# Autodesk Inventor assembly: złożenie gąsienicy lewej
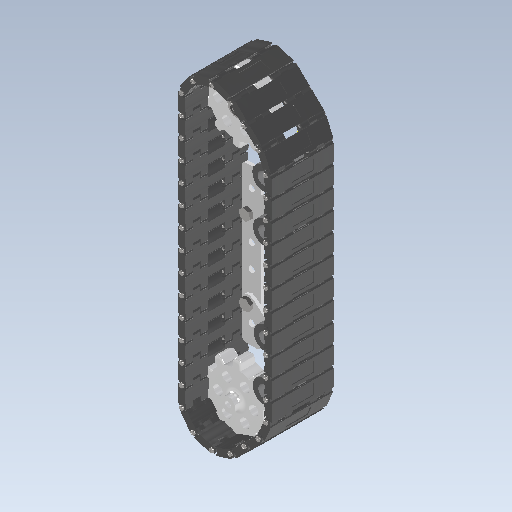
[picture p0: Inventor's stored thumbnail of the model, 512x512]
Saved by Autodesk Inventor 2021 (Build 250183000, 183)
## iProperties
Created: 2021-06-19
Part Number: złożenie gąsienicy lewej
Document SubType Name: Assembly
Designer: Łukasz
Author: Łukasz
## Documents named in this file (14)
- E:\GITHUB_Czołg\Szybki-Czolg-antyRadziecki\złożenie gąsienicy lewej.iam
- E:\GITHUB_Czołg\Szybki-Czolg-antyRadziecki\gąsienica.ipt
- E:\GITHUB_Czołg\Szybki-Czolg-antyRadziecki\koło napędowe.ipt
- E:\GITHUB_Czołg\Szybki-Czolg-antyRadziecki\koło łożyskowane.ipt
- E:\GITHUB_Czołg\Szybki-Czolg-antyRadziecki\dystans łożyska.ipt
- E:\GITHUB_Czołg\Szybki-Czolg-antyRadziecki\mocowanie zawieszenia.ipt
- C:\Users\Łukasz\Documents\Inventor\Content Center Files\R2021\en-US\BS EN ISO 7045 H\EN ISO 7045 - M3 x 30 - 4.8 - H(1).ipt
- E:\GITHUB_Czołg\Szybki-Czolg-antyRadziecki\zawieszenie ramie.ipt
- C:\Users\Łukasz\Documents\Inventor\Content Center Files\R2021\en-US\BS 292 (I)\BS 292 Part 1 - 608 - 8 x 22 x 7.ipt
- E:\GITHUB_Czołg\Szybki-Czolg-antyRadziecki\zawieszenie ramie 2.ipt
- C:\Users\Łukasz\Documents\Inventor\Content Center Files\R2021\en-US\BS EN ISO 4017\BS EN ISO 4017 - M8 x 20BS EN.ipt
- C:\Users\Łukasz\Documents\Inventor\Content Center Files\R2021\en-US\AS 1112 (2)\AS 1112 - M8  Type 8.ipt
- C:\Users\Łukasz\Documents\Inventor\Content Center Files\R2021\en-US\AS 1427(02)\AS 1427 - M8 x 25(2).ipt
- E:\GITHUB_Czołg\Szybki-Czolg-antyRadziecki\kółko zawieszenia.ipt
## Components (153 placed, 13 different names)
1. gąsienica:1 — Rotational:1, Angle:1, Rotational:6, Angle:6, Rotational:66, Rotational:77
2. gąsienica:2 — Rotational:1, Angle:1, Rotational:2, Angle:2, Flush:4, Rotational:65, Rotational:78
3. gąsienica:3 — Rotational:5, Angle:5, Rotational:7, Angle:8, Rotational:61, Rotational:82
4. gąsienica:4 — Rotational:3, Angle:3, Rotational:4, Angle:4, Rotational:63, Rotational:80
5. gąsienica:5 — Rotational:2, Angle:2, Rotational:3, Angle:3, Mate:1, Flush:1, Rotational:64, Rotational:79
6. gąsienica:6 — Rotational:6, Angle:6, Rotational:9, Angle:7, Rotational:67, Rotational:76
7. gąsienica:7 — Rotational:4, Angle:4, Rotational:5, Angle:5, Rotational:62, Rotational:81
8. gąsienica:8 — Rotational:7, Rotational:8, Angle:8, Angle:9, Rotational:60, Rotational:83
9. gąsienica:9 — Rotational:8, Angle:9, Rotational:31, Angle:28, Rotational:59, Rotational:84
10. gąsienica:10 — Rotational:9, Angle:7, Rotational:10, Angle:10, Rotational:68, Rotational:113
11. koło napędowe:1 — Mate:1, Flush:1, Flush:3, Mate:2, Mate:3, Flush:4, Flush:5, Flush:6, Mate:4
12. koło łożyskowane:1 — Flush:3, Mate:2, Mate:3, Insert:1, Insert:2, Insert:3
13. dystans łożyska:1 — Insert:1
14. BS 292: Part 1 (I) (Metric) 608 - 8 x 22 x 7:13 — Insert:2
15. BS 292: Part 1 (I) (Metric) 608 - 8 x 22 x 7:14 — Insert:3
16. gąsienica:11 — Rotational:10, Rotational:11, Angle:10, Angle:11, Rotational:69, Rotational:112
17. gąsienica:12 — Rotational:11, Angle:11, Rotational:12, Angle:12, Rotational:71, Rotational:111
18. gąsienica:13 — Rotational:13, Rotational:14, Angle:13, Angle:14, Rotational:72, Rotational:109
19. gąsienica:14 — Rotational:14, Angle:14, Rotational:15, Angle:15, Rotational:73, Rotational:108
20. gąsienica:15 — Rotational:15, Rotational:16, Angle:15, Angle:16, Rotational:74, Rotational:107
21. gąsienica:16 — Rotational:12, Rotational:13, Angle:12, Angle:13, Rotational:70, Rotational:110
22. gąsienica:17 — Rotational:16, Angle:16, Rotational:17, Angle:17, Rotational:75, Rotational:106
23. gąsienica:18 — Rotational:17, Rotational:18, Angle:17, Angle:18, Rotational:41, Rotational:105
24. gąsienica:19 — Rotational:18, Angle:18, Rotational:19, Angle:19, Rotational:40, Rotational:104
25. gąsienica:20 — Rotational:19, Rotational:20, Angle:19, Angle:20, Rotational:39, Rotational:103
26. gąsienica:21 — Rotational:20, Angle:20, Rotational:21, Angle:21, Rotational:42, Rotational:102
27. gąsienica:22 — Rotational:21, Rotational:22, Angle:21, Angle:22, Rotational:43, Rotational:101
28. gąsienica:23 — Rotational:22, Angle:22, Rotational:23, Angle:23, Rotational:44, Rotational:100
29. gąsienica:24 — Rotational:23, Rotational:24, Angle:23, Angle:24, Rotational:45, Rotational:99
30. gąsienica:25 — Rotational:24, Angle:24, Rotational:25, Angle:25, Rotational:46, Rotational:114
31. gąsienica:26 — Rotational:25, Rotational:26, Angle:25, Angle:26, Rotational:47, Rotational:96
32. gąsienica:27 — Rotational:26, Rotational:27, Angle:26, Angle:27, Rotational:48, Rotational:95
33. gąsienica:28 — Rotational:27, Angle:27, Rotational:37, Angle:36, Rotational:49, Rotational:94
34. gąsienica:29 — Rotational:29, Angle:30, Rotational:32, Angle:32, Rotational:56
35. gąsienica:30 — Rotational:29, Rotational:30, Angle:29, Angle:30, Rotational:57, Rotational:86
36. gąsienica:31 — Rotational:30, Rotational:31, Angle:28, Angle:29, Rotational:58, Rotational:85
37. gąsienica:32 — Rotational:32, Rotational:33, Angle:31, Angle:32, Rotational:55, Rotational:87
38. gąsienica:33 — Rotational:33, Angle:31, Rotational:34, Angle:33, Rotational:54, Rotational:88, Rotational:89
39. gąsienica:34 — Rotational:34, Rotational:36, Angle:33, Angle:34, Rotational:53, Rotational:90
40. gąsienica:35 — Rotational:35, Angle:35, Rotational:38, Angle:37, Rotational:51
41. gąsienica:36 — Rotational:35, Rotational:36, Angle:34, Angle:35, Rotational:52, Rotational:91
42. gąsienica:37 — Rotational:37, Angle:36, Rotational:38, Angle:37, Rotational:50, Rotational:92, Rotational:93
43. mocowanie zawieszenia:1 — Flush:5, Flush:6, Mate:4, Rotational:116, Rotational:125, Rotational:142, Rotational:144
44. BS EN ISO 7045 H - Metric M3 x 30 - 4.8 - H:1 — Rotational:39
45. BS EN ISO 7045 H - Metric M3 x 30 - 4.8 - H:2 — Rotational:40
46. BS EN ISO 7045 H - Metric M3 x 30 - 4.8 - H:3 — Rotational:83
47. BS EN ISO 7045 H - Metric M3 x 30 - 4.8 - H:4 — Rotational:82
48. BS EN ISO 7045 H - Metric M3 x 30 - 4.8 - H:5 — Rotational:75
49. BS EN ISO 7045 H - Metric M3 x 30 - 4.8 - H:6 — Rotational:74
50. BS EN ISO 7045 H - Metric M3 x 30 - 4.8 - H:7 — Rotational:73
51. BS EN ISO 7045 H - Metric M3 x 30 - 4.8 - H:8 — Rotational:72
52. BS EN ISO 7045 H - Metric M3 x 30 - 4.8 - H:9 — Rotational:71
53. BS EN ISO 7045 H - Metric M3 x 30 - 4.8 - H:10 — Rotational:70
54. BS EN ISO 7045 H - Metric M3 x 30 - 4.8 - H:11 — Rotational:69
55. BS EN ISO 7045 H - Metric M3 x 30 - 4.8 - H:12 — Rotational:68
56. BS EN ISO 7045 H - Metric M3 x 30 - 4.8 - H:13 — Rotational:67
57. BS EN ISO 7045 H - Metric M3 x 30 - 4.8 - H:14 — Rotational:66
58. BS EN ISO 7045 H - Metric M3 x 30 - 4.8 - H:15 — Rotational:65
59. BS EN ISO 7045 H - Metric M3 x 30 - 4.8 - H:16 — Rotational:64
60. BS EN ISO 7045 H - Metric M3 x 30 - 4.8 - H:17 — Rotational:63
61. BS EN ISO 7045 H - Metric M3 x 30 - 4.8 - H:18 — Rotational:62
62. BS EN ISO 7045 H - Metric M3 x 30 - 4.8 - H:19 — Rotational:61
63. BS EN ISO 7045 H - Metric M3 x 30 - 4.8 - H:20 — Rotational:60
64. BS EN ISO 7045 H - Metric M3 x 30 - 4.8 - H:21 — Rotational:59
65. BS EN ISO 7045 H - Metric M3 x 30 - 4.8 - H:22 — Rotational:58
66. BS EN ISO 7045 H - Metric M3 x 30 - 4.8 - H:23 — Rotational:57
67. BS EN ISO 7045 H - Metric M3 x 30 - 4.8 - H:24 — Rotational:56
68. BS EN ISO 7045 H - Metric M3 x 30 - 4.8 - H:25 — Rotational:54
69. BS EN ISO 7045 H - Metric M3 x 30 - 4.8 - H:26 — Rotational:52
70. BS EN ISO 7045 H - Metric M3 x 30 - 4.8 - H:27 — Rotational:53
71. BS EN ISO 7045 H - Metric M3 x 30 - 4.8 - H:28 — Rotational:55
72. BS EN ISO 7045 H - Metric M3 x 30 - 4.8 - H:29 — Rotational:51
73. BS EN ISO 7045 H - Metric M3 x 30 - 4.8 - H:30 — Rotational:50
74. BS EN ISO 7045 H - Metric M3 x 30 - 4.8 - H:31 — Rotational:49
75. BS EN ISO 7045 H - Metric M3 x 30 - 4.8 - H:32 — Rotational:48
76. BS EN ISO 7045 H - Metric M3 x 30 - 4.8 - H:33 — Rotational:47
77. BS EN ISO 7045 H - Metric M3 x 30 - 4.8 - H:34 — Rotational:46
78. BS EN ISO 7045 H - Metric M3 x 30 - 4.8 - H:35 — Rotational:45
79. BS EN ISO 7045 H - Metric M3 x 30 - 4.8 - H:36 — Rotational:44
80. BS EN ISO 7045 H - Metric M3 x 30 - 4.8 - H:37 — Rotational:43
81. BS EN ISO 7045 H - Metric M3 x 30 - 4.8 - H:38 — Rotational:42
82. BS EN ISO 7045 H - Metric M3 x 30 - 4.8 - H:39 — Rotational:41
83. BS EN ISO 7045 H - Metric M3 x 30 - 4.8 - H:40 — Rotational:76
84. BS EN ISO 7045 H - Metric M3 x 30 - 4.8 - H:41 — Rotational:77
85. BS EN ISO 7045 H - Metric M3 x 30 - 4.8 - H:42 — Rotational:78
86. BS EN ISO 7045 H - Metric M3 x 30 - 4.8 - H:43 — Rotational:79
87. BS EN ISO 7045 H - Metric M3 x 30 - 4.8 - H:44 — Rotational:80
88. BS EN ISO 7045 H - Metric M3 x 30 - 4.8 - H:45 — Rotational:81
89. BS EN ISO 7045 H - Metric M3 x 30 - 4.8 - H:46 — Rotational:84
90. BS EN ISO 7045 H - Metric M3 x 30 - 4.8 - H:47 — Rotational:85
91. BS EN ISO 7045 H - Metric M3 x 30 - 4.8 - H:48 — Rotational:86
92. BS EN ISO 7045 H - Metric M3 x 30 - 4.8 - H:49 — Rotational:87
93. BS EN ISO 7045 H - Metric M3 x 30 - 4.8 - H:50 — Rotational:88
94. BS EN ISO 7045 H - Metric M3 x 30 - 4.8 - H:51 — Rotational:89
95. BS EN ISO 7045 H - Metric M3 x 30 - 4.8 - H:52 — Rotational:90
96. BS EN ISO 7045 H - Metric M3 x 30 - 4.8 - H:53 — Rotational:91
97. BS EN ISO 7045 H - Metric M3 x 30 - 4.8 - H:54 — Rotational:92
98. BS EN ISO 7045 H - Metric M3 x 30 - 4.8 - H:55 — Rotational:93
99. BS EN ISO 7045 H - Metric M3 x 30 - 4.8 - H:56 — Rotational:94
100. BS EN ISO 7045 H - Metric M3 x 30 - 4.8 - H:57 — Rotational:95
101. BS EN ISO 7045 H - Metric M3 x 30 - 4.8 - H:58 — Rotational:96
102. BS EN ISO 7045 H - Metric M3 x 30 - 4.8 - H:60 — Rotational:114
103. BS EN ISO 7045 H - Metric M3 x 30 - 4.8 - H:61 — Rotational:99
104. BS EN ISO 7045 H - Metric M3 x 30 - 4.8 - H:62 — Rotational:100
105. BS EN ISO 7045 H - Metric M3 x 30 - 4.8 - H:63 — Rotational:101
106. BS EN ISO 7045 H - Metric M3 x 30 - 4.8 - H:64 — Rotational:102
107. BS EN ISO 7045 H - Metric M3 x 30 - 4.8 - H:65 — Rotational:103
108. BS EN ISO 7045 H - Metric M3 x 30 - 4.8 - H:66 — Rotational:104
109. BS EN ISO 7045 H - Metric M3 x 30 - 4.8 - H:67 — Rotational:105
110. BS EN ISO 7045 H - Metric M3 x 30 - 4.8 - H:68 — Rotational:106
111. BS EN ISO 7045 H - Metric M3 x 30 - 4.8 - H:69 — Rotational:107
112. BS EN ISO 7045 H - Metric M3 x 30 - 4.8 - H:70 — Rotational:108
113. BS EN ISO 7045 H - Metric M3 x 30 - 4.8 - H:71 — Rotational:109
114. BS EN ISO 7045 H - Metric M3 x 30 - 4.8 - H:72 — Rotational:110
115. BS EN ISO 7045 H - Metric M3 x 30 - 4.8 - H:73 — Rotational:113
116. BS EN ISO 7045 H - Metric M3 x 30 - 4.8 - H:74 — Rotational:111
117. BS EN ISO 7045 H - Metric M3 x 30 - 4.8 - H:75 — Rotational:112
118. zawieszenie ramie:1 — Rotational:116, Rotational:117, Rotational:119, Rotational:121
119. zawieszenie ramie:2 — Rotational:118, Rotational:122, Rotational:142, Rotational:143
120. AS 1427 - Metric M8 x 25:1 — Rigid:2
121. BS 292: Part 1 (I) (Metric) 608 - 8 x 22 x 7:5 — Rotational:126, Rigid:6, Rotational:137
122. zawieszenie ramie 2:1 — Rotational:117, Rotational:123, Rotational:126, Rotational:127, Rotational:128, Rotational:129
123. zawieszenie ramie 2:2 — Rotational:118, Rotational:130, Rotational:131, Rotational:132, Rotational:133, Rigid:10
124. BS EN ISO 4017 - Metric M8 x 20:1 — Rotational:119
125. BS EN ISO 4017 - Metric M8 x 20:2 — Rotational:122
126. BS EN ISO 4017 - Metric M8 x 20:3 — Rotational:143
127. BS EN ISO 4017 - Metric M8 x 20:4 — Rotational:121
128. AS 1112 (2) - Metric M8  Type 8:1 — Rigid:10
129. AS 1112 (2) - Metric M8  Type 8:2 — Rotational:125
130. AS 1112 (2) - Metric M8  Type 8:3 — Rotational:144
131. AS 1112 (2) - Metric M8  Type 8:4 — Rotational:123
132. BS 292: Part 1 (I) (Metric) 608 - 8 x 22 x 7:6 — Rotational:127, Rigid:7, Rotational:136
133. BS 292: Part 1 (I) (Metric) 608 - 8 x 22 x 7:7 — Rotational:129, Rigid:2, Rotational:141
134. BS 292: Part 1 (I) (Metric) 608 - 8 x 22 x 7:8 — Rotational:128, Rigid:3, Rotational:140
135. BS 292: Part 1 (I) (Metric) 608 - 8 x 22 x 7:9 — Rotational:130, Rigid:4, Rotational:139
136. BS 292: Part 1 (I) (Metric) 608 - 8 x 22 x 7:10 — Rotational:132, Rigid:8, Rotational:135
137. BS 292: Part 1 (I) (Metric) 608 - 8 x 22 x 7:11 — Rotational:131, Rigid:5, Rotational:138
138. BS 292: Part 1 (I) (Metric) 608 - 8 x 22 x 7:12 — Rotational:133, Rigid:9, Rotational:134
139. AS 1427 - Metric M8 x 25:2 — Rigid:3
140. AS 1427 - Metric M8 x 25:3 — Rigid:4
141. AS 1427 - Metric M8 x 25:4 — Rigid:5
142. AS 1112 (2) - Metric M8  Type 8:5 — Rigid:6
143. AS 1112 (2) - Metric M8  Type 8:6 — Rigid:8
144. AS 1112 (2) - Metric M8  Type 8:7 — Rigid:7
145. AS 1112 (2) - Metric M8  Type 8:8 — Rigid:9
146. kółko zawieszenia:1 — Rotational:134
147. kółko zawieszenia:2 — Rotational:138
148. kółko zawieszenia:3 — Rotational:139
149. kółko zawieszenia:4 — Rotational:141
150. kółko zawieszenia:5 — Rotational:135
151. kółko zawieszenia:6 — Rotational:136
152. kółko zawieszenia:7 — Rotational:137
153. kółko zawieszenia:8 — Rotational:140
## Relationships (196: RevoluteJoint 138, Angle 37, WeldJoint 9, Flush 5, Mate 4, Insert 3)
- Rotational:1 [RevoluteJoint]: gąsienica:1 ↔ gąsienica:2
- Angle:1 (-36 deg): gąsienica:1 ↔ gąsienica:2
- Rotational:2 [RevoluteJoint]: gąsienica:2 ↔ gąsienica:5
- Angle:2 (36 deg): gąsienica:2 ↔ gąsienica:5
- Rotational:3 [RevoluteJoint]: gąsienica:4 ↔ gąsienica:5
- Angle:3 (36 deg): gąsienica:4 ↔ gąsienica:5
- Rotational:4 [RevoluteJoint]: gąsienica:4 ↔ gąsienica:7
- Angle:4 (26 deg): gąsienica:4 ↔ gąsienica:7
- Rotational:5 [RevoluteJoint]: gąsienica:3 ↔ gąsienica:7
- Angle:5 (0 deg): gąsienica:3 ↔ gąsienica:7
- Rotational:6 [RevoluteJoint]: gąsienica:1 ↔ gąsienica:6
- Angle:6 (0 deg): gąsienica:1 ↔ gąsienica:6
- Rotational:7 [RevoluteJoint]: gąsienica:3 ↔ gąsienica:8
- Rotational:8 [RevoluteJoint]: gąsienica:8 ↔ gąsienica:9
- Rotational:9 [RevoluteJoint]: gąsienica:6 ↔ gąsienica:10
- Angle:7 (0 deg): gąsienica:6 ↔ gąsienica:10
- Angle:8 (22.893 deg): gąsienica:3 ↔ gąsienica:8
- Angle:9 (23.107 deg): gąsienica:8 ↔ gąsienica:9
- Mate:1 (1 mm): gąsienica:5 ↔ koło napędowe:1
- Flush:1: gąsienica:5 ↔ koło napędowe:1
- Flush:3: koło napędowe:1 ↔ koło łożyskowane:1
- Mate:2 (-325 mm): koło napędowe:1 ↔ koło łożyskowane:1
- Mate:3: koło napędowe:1 ↔ koło łożyskowane:1
- Insert:1 (8 mm): koło łożyskowane:1 ↔ dystans łożyska:1
- Insert:2: koło łożyskowane:1 ↔ BS 292: Part 1 (I) (Metric) 608 - 8 x 22 x 7:13
- Insert:3: koło łożyskowane:1 ↔ BS 292: Part 1 (I) (Metric) 608 - 8 x 22 x 7:14
- Rotational:10 [RevoluteJoint]: gąsienica:10 ↔ gąsienica:11
- Rotational:11 [RevoluteJoint]: gąsienica:11 ↔ gąsienica:12
- Angle:10 (0 deg): gąsienica:10 ↔ gąsienica:11
- Angle:11 (0 deg): gąsienica:11 ↔ gąsienica:12
- Rotational:12 [RevoluteJoint]: gąsienica:12 ↔ gąsienica:16
- Rotational:13 [RevoluteJoint]: gąsienica:13 ↔ gąsienica:16
- Rotational:14 [RevoluteJoint]: gąsienica:13 ↔ gąsienica:14
- Angle:12 (0 deg): gąsienica:12 ↔ gąsienica:16
- Angle:13 (0 deg): gąsienica:13 ↔ gąsienica:16
- Angle:14 (0 deg): gąsienica:13 ↔ gąsienica:14
- Rotational:15 [RevoluteJoint]: gąsienica:14 ↔ gąsienica:15
- Rotational:16 [RevoluteJoint]: gąsienica:15 ↔ gąsienica:17
- Angle:15 (0 deg): gąsienica:14 ↔ gąsienica:15
- Angle:16 (0 deg): gąsienica:15 ↔ gąsienica:17
- Rotational:17 [RevoluteJoint]: gąsienica:17 ↔ gąsienica:18
- Rotational:18 [RevoluteJoint]: gąsienica:18 ↔ gąsienica:19
- Angle:17 (0 deg): gąsienica:17 ↔ gąsienica:18
- Angle:18 (0 deg): gąsienica:18 ↔ gąsienica:19
- Rotational:19 [RevoluteJoint]: gąsienica:19 ↔ gąsienica:20
- Rotational:20 [RevoluteJoint]: gąsienica:20 ↔ gąsienica:21
- Angle:19 (0 deg): gąsienica:19 ↔ gąsienica:20
- Angle:20 (0 deg): gąsienica:20 ↔ gąsienica:21
- Rotational:21 [RevoluteJoint]: gąsienica:21 ↔ gąsienica:22
- Rotational:22 [RevoluteJoint]: gąsienica:22 ↔ gąsienica:23
- Angle:21 (36 deg): gąsienica:21 ↔ gąsienica:22
- Angle:22 (36 deg): gąsienica:22 ↔ gąsienica:23
- Rotational:23 [RevoluteJoint]: gąsienica:23 ↔ gąsienica:24
- Rotational:24 [RevoluteJoint]: gąsienica:24 ↔ gąsienica:25
- Angle:23 (36 deg): gąsienica:23 ↔ gąsienica:24
- Angle:24 (26 deg): gąsienica:24 ↔ gąsienica:25
- Rotational:25 [RevoluteJoint]: gąsienica:25 ↔ gąsienica:26
- Rotational:26 [RevoluteJoint]: gąsienica:26 ↔ gąsienica:27
- Rotational:27 [RevoluteJoint]: gąsienica:27 ↔ gąsienica:28
- Angle:25 (0 deg): gąsienica:25 ↔ gąsienica:26
- Angle:26 (22.893 deg): gąsienica:26 ↔ gąsienica:27
- Angle:27 (23.107 deg): gąsienica:27 ↔ gąsienica:28
- Rotational:29 [RevoluteJoint]: gąsienica:29 ↔ gąsienica:30
- Rotational:30 [RevoluteJoint]: gąsienica:30 ↔ gąsienica:31
- Rotational:31 [RevoluteJoint]: gąsienica:9 ↔ gąsienica:31
- Angle:28 (0 deg): gąsienica:9 ↔ gąsienica:31
- Angle:29 (0 deg): gąsienica:30 ↔ gąsienica:31
- Angle:30 (0 deg): gąsienica:29 ↔ gąsienica:30
- Rotational:32 [RevoluteJoint]: gąsienica:29 ↔ gąsienica:32
- Rotational:33 [RevoluteJoint]: gąsienica:32 ↔ gąsienica:33
- Angle:31 (0 deg): gąsienica:32 ↔ gąsienica:33
- Angle:32 (0 deg): gąsienica:29 ↔ gąsienica:32
- Rotational:34 [RevoluteJoint]: gąsienica:33 ↔ gąsienica:34
- Rotational:35 [RevoluteJoint]: gąsienica:35 ↔ gąsienica:36
- Rotational:36 [RevoluteJoint]: gąsienica:34 ↔ gąsienica:36
- Angle:33 (0 deg): gąsienica:33 ↔ gąsienica:34
- Angle:34 (0 deg): gąsienica:34 ↔ gąsienica:36
- Angle:35 (0 deg): gąsienica:35 ↔ gąsienica:36
- Rotational:37 [RevoluteJoint]: gąsienica:28 ↔ gąsienica:37
- Angle:36 (0 deg): gąsienica:28 ↔ gąsienica:37
- Rotational:38 [RevoluteJoint]: gąsienica:35 ↔ gąsienica:37
- Angle:37 (0 deg): gąsienica:35 ↔ gąsienica:37
- Flush:4: gąsienica:2 ↔ koło napędowe:1
- Flush:5 (8 mm): koło napędowe:1 ↔ mocowanie zawieszenia:1
- Flush:6 (62.5 mm): koło napędowe:1 ↔ mocowanie zawieszenia:1
- Mate:4: koło napędowe:1 ↔ mocowanie zawieszenia:1
- Rotational:39 [RevoluteJoint] (-1 mm): gąsienica:20 ↔ BS EN ISO 7045 H - Metric M3 x 30 - 4.8 - H:1
- Rotational:40 [RevoluteJoint] (-1 mm): gąsienica:19 ↔ BS EN ISO 7045 H - Metric M3 x 30 - 4.8 - H:2
- Rotational:41 [RevoluteJoint] (-1 mm): gąsienica:18 ↔ BS EN ISO 7045 H - Metric M3 x 30 - 4.8 - H:39
- Rotational:42 [RevoluteJoint] (-1 mm): gąsienica:21 ↔ BS EN ISO 7045 H - Metric M3 x 30 - 4.8 - H:38
- Rotational:43 [RevoluteJoint] (-1 mm): gąsienica:22 ↔ BS EN ISO 7045 H - Metric M3 x 30 - 4.8 - H:37
- Rotational:44 [RevoluteJoint] (-1 mm): gąsienica:23 ↔ BS EN ISO 7045 H - Metric M3 x 30 - 4.8 - H:36
- Rotational:45 [RevoluteJoint] (-1 mm): gąsienica:24 ↔ BS EN ISO 7045 H - Metric M3 x 30 - 4.8 - H:35
- Rotational:46 [RevoluteJoint] (-1 mm): gąsienica:25 ↔ BS EN ISO 7045 H - Metric M3 x 30 - 4.8 - H:34
- Rotational:47 [RevoluteJoint] (-1 mm): gąsienica:26 ↔ BS EN ISO 7045 H - Metric M3 x 30 - 4.8 - H:33
- Rotational:48 [RevoluteJoint] (-1 mm): gąsienica:27 ↔ BS EN ISO 7045 H - Metric M3 x 30 - 4.8 - H:32
- Rotational:49 [RevoluteJoint] (-1 mm): gąsienica:28 ↔ BS EN ISO 7045 H - Metric M3 x 30 - 4.8 - H:31
- Rotational:50 [RevoluteJoint] (-1 mm): gąsienica:37 ↔ BS EN ISO 7045 H - Metric M3 x 30 - 4.8 - H:30
- Rotational:51 [RevoluteJoint] (-1 mm): gąsienica:35 ↔ BS EN ISO 7045 H - Metric M3 x 30 - 4.8 - H:29
- Rotational:52 [RevoluteJoint] (-1 mm): gąsienica:36 ↔ BS EN ISO 7045 H - Metric M3 x 30 - 4.8 - H:26
- Rotational:53 [RevoluteJoint] (-1 mm): gąsienica:34 ↔ BS EN ISO 7045 H - Metric M3 x 30 - 4.8 - H:27
- Rotational:54 [RevoluteJoint] (-1 mm): gąsienica:33 ↔ BS EN ISO 7045 H - Metric M3 x 30 - 4.8 - H:25
- Rotational:55 [RevoluteJoint] (-1 mm): gąsienica:32 ↔ BS EN ISO 7045 H - Metric M3 x 30 - 4.8 - H:28
- Rotational:56 [RevoluteJoint] (-1 mm): gąsienica:29 ↔ BS EN ISO 7045 H - Metric M3 x 30 - 4.8 - H:24
- Rotational:57 [RevoluteJoint] (-1 mm): gąsienica:30 ↔ BS EN ISO 7045 H - Metric M3 x 30 - 4.8 - H:23
- Rotational:58 [RevoluteJoint] (-1 mm): gąsienica:31 ↔ BS EN ISO 7045 H - Metric M3 x 30 - 4.8 - H:22
- Rotational:59 [RevoluteJoint] (-1 mm): gąsienica:9 ↔ BS EN ISO 7045 H - Metric M3 x 30 - 4.8 - H:21
- Rotational:60 [RevoluteJoint] (-1 mm): gąsienica:8 ↔ BS EN ISO 7045 H - Metric M3 x 30 - 4.8 - H:20
- Rotational:61 [RevoluteJoint] (-1 mm): gąsienica:3 ↔ BS EN ISO 7045 H - Metric M3 x 30 - 4.8 - H:19
- Rotational:62 [RevoluteJoint] (-1 mm): gąsienica:7 ↔ BS EN ISO 7045 H - Metric M3 x 30 - 4.8 - H:18
- Rotational:63 [RevoluteJoint] (-1 mm): gąsienica:4 ↔ BS EN ISO 7045 H - Metric M3 x 30 - 4.8 - H:17
- Rotational:64 [RevoluteJoint] (-1 mm): gąsienica:5 ↔ BS EN ISO 7045 H - Metric M3 x 30 - 4.8 - H:16
- Rotational:65 [RevoluteJoint] (-1 mm): gąsienica:2 ↔ BS EN ISO 7045 H - Metric M3 x 30 - 4.8 - H:15
- Rotational:66 [RevoluteJoint] (-1 mm): gąsienica:1 ↔ BS EN ISO 7045 H - Metric M3 x 30 - 4.8 - H:14
- Rotational:67 [RevoluteJoint] (1 mm): gąsienica:6 ↔ BS EN ISO 7045 H - Metric M3 x 30 - 4.8 - H:13
- Rotational:68 [RevoluteJoint] (-1 mm): gąsienica:10 ↔ BS EN ISO 7045 H - Metric M3 x 30 - 4.8 - H:12
- Rotational:69 [RevoluteJoint] (-1 mm): gąsienica:11 ↔ BS EN ISO 7045 H - Metric M3 x 30 - 4.8 - H:11
- Rotational:70 [RevoluteJoint] (-1 mm): gąsienica:16 ↔ BS EN ISO 7045 H - Metric M3 x 30 - 4.8 - H:10
- Rotational:71 [RevoluteJoint] (-1 mm): gąsienica:12 ↔ BS EN ISO 7045 H - Metric M3 x 30 - 4.8 - H:9
- Rotational:72 [RevoluteJoint] (-1 mm): gąsienica:13 ↔ BS EN ISO 7045 H - Metric M3 x 30 - 4.8 - H:8
- Rotational:73 [RevoluteJoint] (-1 mm): gąsienica:14 ↔ BS EN ISO 7045 H - Metric M3 x 30 - 4.8 - H:7
- Rotational:74 [RevoluteJoint] (-1 mm): gąsienica:15 ↔ BS EN ISO 7045 H - Metric M3 x 30 - 4.8 - H:6
- Rotational:75 [RevoluteJoint] (-1 mm): gąsienica:17 ↔ BS EN ISO 7045 H - Metric M3 x 30 - 4.8 - H:5
- Rotational:76 [RevoluteJoint] (-1 mm): gąsienica:6 ↔ BS EN ISO 7045 H - Metric M3 x 30 - 4.8 - H:40
- Rotational:77 [RevoluteJoint] (-1 mm): gąsienica:1 ↔ BS EN ISO 7045 H - Metric M3 x 30 - 4.8 - H:41
- Rotational:78 [RevoluteJoint] (-1 mm): gąsienica:2 ↔ BS EN ISO 7045 H - Metric M3 x 30 - 4.8 - H:42
- Rotational:79 [RevoluteJoint] (-1 mm): gąsienica:5 ↔ BS EN ISO 7045 H - Metric M3 x 30 - 4.8 - H:43
- Rotational:80 [RevoluteJoint] (-1 mm): gąsienica:4 ↔ BS EN ISO 7045 H - Metric M3 x 30 - 4.8 - H:44
- Rotational:81 [RevoluteJoint] (-1 mm): gąsienica:7 ↔ BS EN ISO 7045 H - Metric M3 x 30 - 4.8 - H:45
- Rotational:82 [RevoluteJoint] (-1 mm): gąsienica:3 ↔ BS EN ISO 7045 H - Metric M3 x 30 - 4.8 - H:4
- Rotational:83 [RevoluteJoint] (-1 mm): gąsienica:8 ↔ BS EN ISO 7045 H - Metric M3 x 30 - 4.8 - H:3
- Rotational:84 [RevoluteJoint] (-1 mm): gąsienica:9 ↔ BS EN ISO 7045 H - Metric M3 x 30 - 4.8 - H:46
- Rotational:85 [RevoluteJoint] (-1 mm): gąsienica:31 ↔ BS EN ISO 7045 H - Metric M3 x 30 - 4.8 - H:47
- Rotational:86 [RevoluteJoint] (-1 mm): gąsienica:30 ↔ BS EN ISO 7045 H - Metric M3 x 30 - 4.8 - H:48
- Rotational:87 [RevoluteJoint] (-1 mm): gąsienica:32 ↔ BS EN ISO 7045 H - Metric M3 x 30 - 4.8 - H:49
- Rotational:88 [RevoluteJoint] (-1 mm): gąsienica:33 ↔ BS EN ISO 7045 H - Metric M3 x 30 - 4.8 - H:50
- Rotational:89 [RevoluteJoint] (-1 mm): gąsienica:33 ↔ BS EN ISO 7045 H - Metric M3 x 30 - 4.8 - H:51
- Rotational:90 [RevoluteJoint] (1 mm): gąsienica:34 ↔ BS EN ISO 7045 H - Metric M3 x 30 - 4.8 - H:52
- Rotational:91 [RevoluteJoint] (-1 mm): gąsienica:36 ↔ BS EN ISO 7045 H - Metric M3 x 30 - 4.8 - H:53
- Rotational:92 [RevoluteJoint] (-1 mm): gąsienica:37 ↔ BS EN ISO 7045 H - Metric M3 x 30 - 4.8 - H:54
- Rotational:93 [RevoluteJoint] (-1 mm): gąsienica:37 ↔ BS EN ISO 7045 H - Metric M3 x 30 - 4.8 - H:55
- Rotational:94 [RevoluteJoint] (1 mm): gąsienica:28 ↔ BS EN ISO 7045 H - Metric M3 x 30 - 4.8 - H:56
- Rotational:95 [RevoluteJoint] (-1 mm): gąsienica:27 ↔ BS EN ISO 7045 H - Metric M3 x 30 - 4.8 - H:57
- Rotational:96 [RevoluteJoint] (-1 mm): gąsienica:26 ↔ BS EN ISO 7045 H - Metric M3 x 30 - 4.8 - H:58
- Rotational:99 [RevoluteJoint] (-1 mm): gąsienica:24 ↔ BS EN ISO 7045 H - Metric M3 x 30 - 4.8 - H:61
- Rotational:100 [RevoluteJoint] (1 mm): gąsienica:23 ↔ BS EN ISO 7045 H - Metric M3 x 30 - 4.8 - H:62
- Rotational:101 [RevoluteJoint] (-1 mm): gąsienica:22 ↔ BS EN ISO 7045 H - Metric M3 x 30 - 4.8 - H:63
- Rotational:102 [RevoluteJoint] (-1 mm): gąsienica:21 ↔ BS EN ISO 7045 H - Metric M3 x 30 - 4.8 - H:64
- Rotational:103 [RevoluteJoint] (-1 mm): gąsienica:20 ↔ BS EN ISO 7045 H - Metric M3 x 30 - 4.8 - H:65
- Rotational:104 [RevoluteJoint] (-1 mm): gąsienica:19 ↔ BS EN ISO 7045 H - Metric M3 x 30 - 4.8 - H:66
- Rotational:105 [RevoluteJoint] (-1 mm): gąsienica:18 ↔ BS EN ISO 7045 H - Metric M3 x 30 - 4.8 - H:67
- Rotational:106 [RevoluteJoint] (-1 mm): gąsienica:17 ↔ BS EN ISO 7045 H - Metric M3 x 30 - 4.8 - H:68
- Rotational:107 [RevoluteJoint] (-1 mm): gąsienica:15 ↔ BS EN ISO 7045 H - Metric M3 x 30 - 4.8 - H:69
- Rotational:108 [RevoluteJoint] (-1 mm): gąsienica:14 ↔ BS EN ISO 7045 H - Metric M3 x 30 - 4.8 - H:70
- Rotational:109 [RevoluteJoint] (-1 mm): gąsienica:13 ↔ BS EN ISO 7045 H - Metric M3 x 30 - 4.8 - H:71
- Rotational:110 [RevoluteJoint] (-1 mm): gąsienica:16 ↔ BS EN ISO 7045 H - Metric M3 x 30 - 4.8 - H:72
- Rotational:111 [RevoluteJoint] (-1 mm): gąsienica:12 ↔ BS EN ISO 7045 H - Metric M3 x 30 - 4.8 - H:74
- Rotational:112 [RevoluteJoint] (-1 mm): gąsienica:11 ↔ BS EN ISO 7045 H - Metric M3 x 30 - 4.8 - H:75
- Rotational:113 [RevoluteJoint] (-1 mm): gąsienica:10 ↔ BS EN ISO 7045 H - Metric M3 x 30 - 4.8 - H:73
- Rotational:114 [RevoluteJoint] (-1 mm): gąsienica:25 ↔ BS EN ISO 7045 H - Metric M3 x 30 - 4.8 - H:60
- Rotational:116 [RevoluteJoint]: mocowanie zawieszenia:1 ↔ zawieszenie ramie:1
- Rotational:117 [RevoluteJoint]: zawieszenie ramie:1 ↔ zawieszenie ramie 2:1
- Rotational:118 [RevoluteJoint]: zawieszenie ramie:2 ↔ zawieszenie ramie 2:2
- Rotational:119 [RevoluteJoint]: zawieszenie ramie:1 ↔ BS EN ISO 4017 - Metric M8 x 20:1
- Rotational:121 [RevoluteJoint]: zawieszenie ramie:1 ↔ BS EN ISO 4017 - Metric M8 x 20:4
- Rotational:122 [RevoluteJoint]: zawieszenie ramie:2 ↔ BS EN ISO 4017 - Metric M8 x 20:2
- Rotational:123 [RevoluteJoint]: zawieszenie ramie 2:1 ↔ AS 1112 (2) - Metric M8  Type 8:4
- Rotational:125 [RevoluteJoint]: mocowanie zawieszenia:1 ↔ AS 1112 (2) - Metric M8  Type 8:2
- Rotational:126 [RevoluteJoint]: BS 292: Part 1 (I) (Metric) 608 - 8 x 22 x 7:5 ↔ zawieszenie ramie 2:1
- Rotational:127 [RevoluteJoint]: zawieszenie ramie 2:1 ↔ BS 292: Part 1 (I) (Metric) 608 - 8 x 22 x 7:6
- Rotational:128 [RevoluteJoint]: zawieszenie ramie 2:1 ↔ BS 292: Part 1 (I) (Metric) 608 - 8 x 22 x 7:8
- Rotational:129 [RevoluteJoint]: zawieszenie ramie 2:1 ↔ BS 292: Part 1 (I) (Metric) 608 - 8 x 22 x 7:7
- Rotational:130 [RevoluteJoint]: zawieszenie ramie 2:2 ↔ BS 292: Part 1 (I) (Metric) 608 - 8 x 22 x 7:9
- Rotational:131 [RevoluteJoint]: zawieszenie ramie 2:2 ↔ BS 292: Part 1 (I) (Metric) 608 - 8 x 22 x 7:11
- Rotational:132 [RevoluteJoint]: zawieszenie ramie 2:2 ↔ BS 292: Part 1 (I) (Metric) 608 - 8 x 22 x 7:10
- Rotational:133 [RevoluteJoint]: zawieszenie ramie 2:2 ↔ BS 292: Part 1 (I) (Metric) 608 - 8 x 22 x 7:12
- Rigid:2 [WeldJoint]: AS 1427 - Metric M8 x 25:1 ↔ BS 292: Part 1 (I) (Metric) 608 - 8 x 22 x 7:7
- Rigid:3 [WeldJoint]: BS 292: Part 1 (I) (Metric) 608 - 8 x 22 x 7:8 ↔ AS 1427 - Metric M8 x 25:2
- Rigid:4 [WeldJoint]: BS 292: Part 1 (I) (Metric) 608 - 8 x 22 x 7:9 ↔ AS 1427 - Metric M8 x 25:3
- Rigid:5 [WeldJoint]: BS 292: Part 1 (I) (Metric) 608 - 8 x 22 x 7:11 ↔ AS 1427 - Metric M8 x 25:4
- Rigid:6 [WeldJoint]: BS 292: Part 1 (I) (Metric) 608 - 8 x 22 x 7:5 ↔ AS 1112 (2) - Metric M8  Type 8:5
- Rigid:7 [WeldJoint]: BS 292: Part 1 (I) (Metric) 608 - 8 x 22 x 7:6 ↔ AS 1112 (2) - Metric M8  Type 8:7
- Rigid:8 [WeldJoint]: BS 292: Part 1 (I) (Metric) 608 - 8 x 22 x 7:10 ↔ AS 1112 (2) - Metric M8  Type 8:6
- Rigid:9 [WeldJoint]: BS 292: Part 1 (I) (Metric) 608 - 8 x 22 x 7:12 ↔ AS 1112 (2) - Metric M8  Type 8:8
- Rotational:134 [RevoluteJoint]: BS 292: Part 1 (I) (Metric) 608 - 8 x 22 x 7:12 ↔ kółko zawieszenia:1
- Rotational:135 [RevoluteJoint]: BS 292: Part 1 (I) (Metric) 608 - 8 x 22 x 7:10 ↔ kółko zawieszenia:5
- Rotational:136 [RevoluteJoint]: BS 292: Part 1 (I) (Metric) 608 - 8 x 22 x 7:6 ↔ kółko zawieszenia:6
- Rotational:137 [RevoluteJoint]: BS 292: Part 1 (I) (Metric) 608 - 8 x 22 x 7:5 ↔ kółko zawieszenia:7
- Rotational:138 [RevoluteJoint]: BS 292: Part 1 (I) (Metric) 608 - 8 x 22 x 7:11 ↔ kółko zawieszenia:2
- Rotational:139 [RevoluteJoint]: BS 292: Part 1 (I) (Metric) 608 - 8 x 22 x 7:9 ↔ kółko zawieszenia:3
- Rotational:140 [RevoluteJoint]: BS 292: Part 1 (I) (Metric) 608 - 8 x 22 x 7:8 ↔ kółko zawieszenia:8
- Rotational:141 [RevoluteJoint]: BS 292: Part 1 (I) (Metric) 608 - 8 x 22 x 7:7 ↔ kółko zawieszenia:4
- Rotational:142 [RevoluteJoint]: mocowanie zawieszenia:1 ↔ zawieszenie ramie:2
- Rotational:143 [RevoluteJoint]: zawieszenie ramie:2 ↔ BS EN ISO 4017 - Metric M8 x 20:3
- Rotational:144 [RevoluteJoint]: mocowanie zawieszenia:1 ↔ AS 1112 (2) - Metric M8  Type 8:3
- Rigid:10 [WeldJoint]: zawieszenie ramie 2:2 ↔ AS 1112 (2) - Metric M8  Type 8:1
